# Autodesk Inventor assembly: Ensamble eléctrico
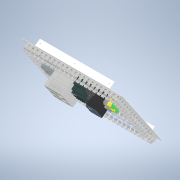
[picture p0: Inventor's stored thumbnail of the model, 180x180]
Saved by Autodesk Inventor 2021 (Build 250183000, 183)
## iProperties
Created: 2021-04-14
Part Number: Ensamble eléctrico
Document SubType Name: Assembly
Designer: Nelson
Author: Nelson
## Documents named in this file (16)
- C:\Users\Nelson\Github\Proyecto_PAI_2021\01 CAD\Ensamble eléctrico.iam
- D:\Nelson\Documentos\Inventor\Proyecto_PAI\PLC-CP1E_N20DT1_D.iam
- D:\Nelson\Documentos\Inventor\Proyecto_PAI\FuenteDC.iam
- D:\Nelson\Documentos\Inventor\Proyecto_PAI\Rele de estado solido.ipt
- D:\Nelson\Documentos\Inventor\Proyecto_PAI\Portafusible para fusible de 2A.ipt
- D:\Nelson\Documentos\Inventor\Proyecto_PAI\Bobina_Electrovalvula.iam
- D:\Nelson\Documentos\Inventor\Proyecto_PAI\Electrovalvula-5_2.ipt
- D:\Nelson\Documentos\Inventor\Proyecto_PAI\Contactor.ipt
- D:\Nelson\Documentos\Inventor\Proyecto_PAI\Riel 35x7.5 378mm.ipt
- D:\Nelson\Documentos\Inventor\Proyecto_PAI\Bornera_AC.ipt
- D:\Nelson\Documentos\Inventor\Proyecto_PAI\Bornera_DC.ipt
- D:\Nelson\Documentos\Inventor\Proyecto_PAI\Bornera_Tierra.ipt
- D:\Nelson\Documentos\Inventor\Proyecto_PAI\Canaleta 30x30 438mm.iam
- D:\Nelson\Documentos\Inventor\Proyecto_PAI\Canaleta 30x30 378mm.iam
- D:\Nelson\Documentos\Inventor\Proyecto_PAI\Canaleta 30x30 317mm.iam
- C:\Users\Nelson\Github\Proyecto_PAI_2021\01 CAD\Tapa_interior_1b.ipt
## Components (31 placed, 15 different names)
1. PLC-CP1E_N20DT1_D:1 [sub-assembly] — Mate:13, Mate:14, Mate:76, Mate:90
2. FuenteDC:1 [sub-assembly] — Mate:15, Mate:16, Mate:62, Mate:76
3. Portafusible para fusible de 2A:1 — Mate:17, Mate:18, Mate:62, Mate:63
4. Bobina_Electrovalvula:1 [sub-assembly] — Mate:9, Flush:13, Flush:14
5. Electrovalvula-5_2:1 — Mate:9, Flush:13, Flush:14, Mate:98, Mate:99, Mate:102, Flush:50
6. Contactor:1 — Mate:19, Mate:20, Mate:63, Mate:64
7. Riel 35x7.5 378mm:1 — Mate:13, Mate:14, Mate:15, Mate:16, Mate:17, Mate:18, Mate:19, Mate:20, Mate:21, Mate:22, Mate:23, Mate:24, Mate:26, Mate:27, Mate:28, Mate:29, Mate:31, Mate:32, Mate:34, Mate:35, Mate:37, Mate:38, Mate:39, Mate:40, Mate:42, Mate:43, Mate:45, Mate:46, Mate:48, Mate:49, Mate:51, Mate:52, Mate:53, Mate:54, Mate:56, Mate:57, Mate:87, Mate:96, Mate:97, Flush:45
8. Bornera_AC:1 — Mate:21, Mate:22, Mate:25, Mate:64
9. Bornera_AC:2 — Mate:23, Mate:24, Mate:25, Mate:65
10. Bornera_DC:1 — Mate:26, Mate:27, Mate:30, Mate:89
11. Bornera_DC:2 — Mate:28, Mate:29, Mate:30, Mate:33
12. Bornera_DC:3 — Mate:31, Mate:32, Mate:33, Mate:36
13. Bornera_DC:4 — Mate:34, Mate:35, Mate:36, Mate:88
14. Bornera_DC:5 — Mate:39, Mate:40, Mate:41, Mate:44
15. Bornera_DC:6 — Mate:42, Mate:43, Mate:44, Mate:47
16. Bornera_DC:7 — Mate:45, Mate:46, Mate:47, Mate:50
17. Bornera_DC:8 — Mate:48, Mate:49, Mate:50, Mate:89
18. Bornera_DC:9 — Mate:37, Mate:38, Mate:41, Mate:90
19. Bornera_Tierra:1 — Mate:51, Mate:52, Mate:55, Mate:65
20. Bornera_Tierra:2 — Mate:53, Mate:54, Mate:55, Mate:58
21. Bornera_Tierra:3 — Mate:56, Mate:57, Mate:58
22. Canaleta 30x30 438mm:1 [sub-assembly] — Mate:79, Mate:83, Mate:96, Mate:109, Flush:41, Flush:52
23. Canaleta 30x30 317mm:1 [sub-assembly] — Mate:79, Mate:81, Mate:87, Mate:88, Mate:94, Mate:99, Flush:41, Flush:42, Flush:51
24. Canaleta 30x30 438mm:2 [sub-assembly] — Mate:81, Mate:84, Flush:42, Flush:43
25. Canaleta 30x30 317mm:2 [sub-assembly] — Mate:83, Mate:84, Flush:43, Flush:44, Flush:45
26. Canaleta 30x30 378mm:1 [sub-assembly] — Mate:94, Mate:97, Mate:98, Mate:101, Flush:44, Flush:49, Flush:50
27. Rele de estado solido:1 — Mate:101, Mate:102, Flush:38, Mate:104, Flush:46, Flush:49
28. Rele de estado solido:2 — Flush:38, Mate:104, Flush:39, Mate:106, Flush:46, Flush:47
29. Rele de estado solido:3 — Flush:39, Mate:106, Flush:40, Mate:108, Flush:47, Flush:48
30. Rele de estado solido:4 — Flush:40, Mate:108, Flush:48
31. Tapa_interior_1b:1 — Mate:109, Flush:51, Flush:52
## Relationships (88: Mate 71, Flush 17)
- Mate:9: Bobina_Electrovalvula:1 ↔ Electrovalvula-5_2:1
- Flush:13: Bobina_Electrovalvula:1 ↔ Electrovalvula-5_2:1
- Flush:14: Bobina_Electrovalvula:1 ↔ Electrovalvula-5_2:1
- Mate:13: PLC-CP1E_N20DT1_D:1 ↔ Riel 35x7.5 378mm:1
- Mate:14: PLC-CP1E_N20DT1_D:1 ↔ Riel 35x7.5 378mm:1
- Mate:15: FuenteDC:1 ↔ Riel 35x7.5 378mm:1
- Mate:16: FuenteDC:1 ↔ Riel 35x7.5 378mm:1
- Mate:17: Portafusible para fusible de 2A:1 ↔ Riel 35x7.5 378mm:1
- Mate:18: Portafusible para fusible de 2A:1 ↔ Riel 35x7.5 378mm:1
- Mate:19: Contactor:1 ↔ Riel 35x7.5 378mm:1
- Mate:20: Contactor:1 ↔ Riel 35x7.5 378mm:1
- Mate:21: Riel 35x7.5 378mm:1 ↔ Bornera_AC:1
- Mate:22: Riel 35x7.5 378mm:1 ↔ Bornera_AC:1
- Mate:23: Riel 35x7.5 378mm:1 ↔ Bornera_AC:2
- Mate:24: Riel 35x7.5 378mm:1 ↔ Bornera_AC:2
- Mate:25: Bornera_AC:1 ↔ Bornera_AC:2
- Mate:26: Riel 35x7.5 378mm:1 ↔ Bornera_DC:1
- Mate:27: Riel 35x7.5 378mm:1 ↔ Bornera_DC:1
- Mate:28: Riel 35x7.5 378mm:1 ↔ Bornera_DC:2
- Mate:29: Riel 35x7.5 378mm:1 ↔ Bornera_DC:2
- Mate:30: Bornera_DC:1 ↔ Bornera_DC:2
- Mate:31: Riel 35x7.5 378mm:1 ↔ Bornera_DC:3
- Mate:32: Riel 35x7.5 378mm:1 ↔ Bornera_DC:3
- Mate:33: Bornera_DC:2 ↔ Bornera_DC:3
- Mate:34: Riel 35x7.5 378mm:1 ↔ Bornera_DC:4
- Mate:35: Riel 35x7.5 378mm:1 ↔ Bornera_DC:4
- Mate:36: Bornera_DC:3 ↔ Bornera_DC:4
- Mate:37: Riel 35x7.5 378mm:1 ↔ Bornera_DC:9
- Mate:38: Riel 35x7.5 378mm:1 ↔ Bornera_DC:9
- Mate:39: Riel 35x7.5 378mm:1 ↔ Bornera_DC:5
- Mate:40: Riel 35x7.5 378mm:1 ↔ Bornera_DC:5
- Mate:41: Bornera_DC:5 ↔ Bornera_DC:9
- Mate:42: Riel 35x7.5 378mm:1 ↔ Bornera_DC:6
- Mate:43: Riel 35x7.5 378mm:1 ↔ Bornera_DC:6
- Mate:44: Bornera_DC:5 ↔ Bornera_DC:6
- Mate:45: Riel 35x7.5 378mm:1 ↔ Bornera_DC:7
- Mate:46: Riel 35x7.5 378mm:1 ↔ Bornera_DC:7
- Mate:47: Bornera_DC:6 ↔ Bornera_DC:7
- Mate:48: Riel 35x7.5 378mm:1 ↔ Bornera_DC:8
- Mate:49: Riel 35x7.5 378mm:1 ↔ Bornera_DC:8
- Mate:50: Bornera_DC:7 ↔ Bornera_DC:8
- Mate:51: Riel 35x7.5 378mm:1 ↔ Bornera_Tierra:1
- Mate:52: Riel 35x7.5 378mm:1 ↔ Bornera_Tierra:1
- Mate:53: Riel 35x7.5 378mm:1 ↔ Bornera_Tierra:2
- Mate:54: Riel 35x7.5 378mm:1 ↔ Bornera_Tierra:2
- Mate:55: Bornera_Tierra:1 ↔ Bornera_Tierra:2
- Mate:56: Riel 35x7.5 378mm:1 ↔ Bornera_Tierra:3
- Mate:57: Riel 35x7.5 378mm:1 ↔ Bornera_Tierra:3
- Mate:58: Bornera_Tierra:2 ↔ Bornera_Tierra:3
- Mate:62 (7 mm): FuenteDC:1 ↔ Portafusible para fusible de 2A:1
- Mate:63 (7 mm): Portafusible para fusible de 2A:1 ↔ Contactor:1
- Mate:64 (7 mm): Contactor:1 ↔ Bornera_AC:1
- Mate:65 (7 mm): Bornera_AC:2 ↔ Bornera_Tierra:1
- Mate:76 (7 mm): PLC-CP1E_N20DT1_D:1 ↔ FuenteDC:1
- Mate:79: Canaleta 30x30 438mm:1 ↔ Canaleta 30x30 317mm:1
- Mate:81: Canaleta 30x30 317mm:1 ↔ Canaleta 30x30 438mm:2
- Mate:83: Canaleta 30x30 438mm:1 ↔ Canaleta 30x30 317mm:2
- Mate:84: Canaleta 30x30 438mm:2 ↔ Canaleta 30x30 317mm:2
- Mate:87: Riel 35x7.5 378mm:1 ↔ Canaleta 30x30 317mm:1
- Mate:88 (24 mm): Bornera_DC:4 ↔ Canaleta 30x30 317mm:1
- Mate:89 (7 mm): Bornera_DC:1 ↔ Bornera_DC:8
- Mate:90 (7 mm): PLC-CP1E_N20DT1_D:1 ↔ Bornera_DC:9
- Mate:94: Canaleta 30x30 317mm:1 ↔ Canaleta 30x30 378mm:1
- Mate:96 (47 mm): Riel 35x7.5 378mm:1 ↔ Canaleta 30x30 438mm:1
- Mate:97 (48 mm): Riel 35x7.5 378mm:1 ↔ Canaleta 30x30 378mm:1
- Mate:98 (26 mm): Electrovalvula-5_2:1 ↔ Canaleta 30x30 378mm:1
- Mate:99 (75 mm): Electrovalvula-5_2:1 ↔ Canaleta 30x30 317mm:1
- Mate:101 (23 mm): Canaleta 30x30 378mm:1 ↔ Rele de estado solido:1
- Mate:102 (10 mm): Electrovalvula-5_2:1 ↔ Rele de estado solido:1
- Flush:38: Rele de estado solido:1 ↔ Rele de estado solido:2
- Mate:104 (9 mm): Rele de estado solido:1 ↔ Rele de estado solido:2
- Flush:39: Rele de estado solido:2 ↔ Rele de estado solido:3
- Mate:106 (9 mm): Rele de estado solido:2 ↔ Rele de estado solido:3
- Flush:40: Rele de estado solido:3 ↔ Rele de estado solido:4
- Mate:108 (9 mm): Rele de estado solido:3 ↔ Rele de estado solido:4
- Mate:109: Canaleta 30x30 438mm:1 ↔ Tapa_interior_1b:1
- Flush:41: Canaleta 30x30 438mm:1 ↔ Canaleta 30x30 317mm:1
- Flush:42: Canaleta 30x30 317mm:1 ↔ Canaleta 30x30 438mm:2
- Flush:43: Canaleta 30x30 438mm:2 ↔ Canaleta 30x30 317mm:2
- Flush:44: Canaleta 30x30 317mm:2 ↔ Canaleta 30x30 378mm:1
- Flush:45: Riel 35x7.5 378mm:1 ↔ Canaleta 30x30 317mm:2
- Flush:46: Rele de estado solido:1 ↔ Rele de estado solido:2
- Flush:47: Rele de estado solido:2 ↔ Rele de estado solido:3
- Flush:48: Rele de estado solido:3 ↔ Rele de estado solido:4
- Flush:49: Canaleta 30x30 378mm:1 ↔ Rele de estado solido:1
- Flush:50: Electrovalvula-5_2:1 ↔ Canaleta 30x30 378mm:1
- Flush:51 (23 mm): Canaleta 30x30 317mm:1 ↔ Tapa_interior_1b:1
- Flush:52 (10 mm): Canaleta 30x30 438mm:1 ↔ Tapa_interior_1b:1
